# Autodesk Inventor assembly: Bed Assembly
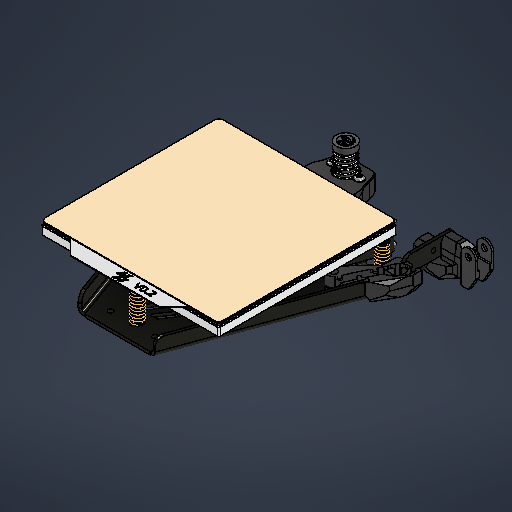
[picture p0: Inventor's stored thumbnail of the model, 512x512]
Saved by Autodesk Inventor 2026 (Build 300175050, 175E)
## iProperties
Created: 2025-05-09
Part Number: Bed Assembly
Document SubType Name: Assembly
Designer: AdminForWorker
Title: Bed Assembly
Author: AdminForWorker
## Documents named in this file (10)
- C:\Users\Joshua Eah\Documents\GitHub\Voron-0\CAD\Master Assembly\Z Axis\Bed Assembly.iam
- C:\Users\Joshua Eah\Documents\GitHub\Voron-0\CAD\Master Assembly\Z Axis\Subassemblies\Build Plate.iam
- C:\Users\Joshua Eah\Documents\GitHub\Voron-0\CAD\Master Assembly\Z Axis\Subassemblies\Kirigami Bed.iam
- C:\Users\Joshua Eah\Documents\GitHub\Voron-0\CAD\Master Assembly\Hardware\M3x16 BHCS.ipt
- C:\Users\Joshua Eah\Documents\GitHub\Voron-0\CAD\Master Assembly\Hardware\M3x40 BHCS.ipt
- C:\Users\Joshua Eah\Documents\GitHub\Voron-0\CAD\Master Assembly\Hardware\M3x12 BHCS.ipt
- C:\Users\Joshua Eah\Documents\GitHub\Voron-0\CAD\Master Assembly\Z Axis\Parts\TR8x8 Antibacklash Nut.ipt
- C:\Users\Joshua Eah\Documents\GitHub\Voron-0\CAD\Master Assembly\Z Axis\Subassemblies\Bed Leveling Screw.iam
- C:\Users\Joshua Eah\Documents\GitHub\Voron-0\CAD\Master Assembly\Z Axis\Subassemblies\Thumb Nut.iam
- C:\Users\Joshua Eah\Documents\GitHub\Voron-0\CAD\Master Assembly\Z Axis\Parts\040-07-12 (1).ipt
## Components (17 placed, 9 different names)
1. Build Plate:1 [sub-assembly] — Insert:7, Insert:8, Insert:9, Insert:10, Insert:11, Insert:12
2. M3x40 BHCS:1 — Insert:7, Mate:5, Mate:8
3. M3x40 BHCS:2 — Insert:8, Mate:9
4. M3x40 BHCS:3 — Insert:9, Mate:7
5. Kirigami Bed:1 [sub-assembly] — Mate:5, Mate:6, Mate:10, Mate:11, Mate:12, Mate:13, Mate:16, Mate:17, Mate:18, Angle:1
6. M3x16 BHCS:1
7. M3x16 BHCS:2
8. M3x12 BHCS:1 — Mate:14, Mate:16
9. M3x12 BHCS:2 — Mate:15, Mate:17
10. TR8x8 Antibacklash Nut:1 — Mate:13, Mate:14, Mate:15, Mate:18, Angle:1
11. Bed Leveling Screw:1 [sub-assembly] — Insert:10, Mate:6
12. Bed Leveling Screw:2 [sub-assembly] — Insert:11
13. Bed Leveling Screw:3 [sub-assembly] — Insert:12
14. Thumb Nut:1 [sub-assembly] — Mate:7, Mate:10
15. Thumb Nut:2 [sub-assembly] — Mate:8, Mate:11
16. Thumb Nut:3 [sub-assembly] — Mate:9, Mate:12
17. 040-07-12 (1):1
## Relationships (26: Mate 15, Insert 10, Angle 1)
- [Mate]: M3x40 BHCS:3 ↔ Kirigami Bed:1
- [Insert]: Kirigami Bed:1 ↔ 040-07-12 (1):1
- [Insert]: Kirigami Bed:1 ↔ 040-07-12 (1):1
- [Insert]: M3x16 BHCS:1 ↔ 040-07-12 (1):1
- [Insert]: M3x16 BHCS:2 ↔ 040-07-12 (1):1
- Insert:7: Build Plate:1 ↔ M3x40 BHCS:1
- Insert:8: Build Plate:1 ↔ M3x40 BHCS:2
- Insert:9: Build Plate:1 ↔ M3x40 BHCS:3
- Insert:10: Build Plate:1 ↔ Bed Leveling Screw:1
- Insert:11: Build Plate:1 ↔ Bed Leveling Screw:2
- Insert:12: Build Plate:1 ↔ Bed Leveling Screw:3
- Mate:5: M3x40 BHCS:1 ↔ Kirigami Bed:1
- Mate:6: Kirigami Bed:1 ↔ Bed Leveling Screw:1
- Mate:7: M3x40 BHCS:3 ↔ Thumb Nut:1
- Mate:8: M3x40 BHCS:1 ↔ Thumb Nut:2
- Mate:9: M3x40 BHCS:2 ↔ Thumb Nut:3
- Mate:10: Kirigami Bed:1 ↔ Thumb Nut:1
- Mate:11: Kirigami Bed:1 ↔ Thumb Nut:2
- Mate:12: Kirigami Bed:1 ↔ Thumb Nut:3
- Mate:13: Kirigami Bed:1 ↔ TR8x8 Antibacklash Nut:1
- Mate:14: M3x12 BHCS:1 ↔ TR8x8 Antibacklash Nut:1
- Mate:15: M3x12 BHCS:2 ↔ TR8x8 Antibacklash Nut:1
- Mate:16: Kirigami Bed:1 ↔ M3x12 BHCS:1
- Mate:17: Kirigami Bed:1 ↔ M3x12 BHCS:2
- Mate:18: Kirigami Bed:1 ↔ TR8x8 Antibacklash Nut:1
- Angle:1 (0 deg): Kirigami Bed:1 ↔ TR8x8 Antibacklash Nut:1
